# Autodesk Inventor assembly: ASY MSC 120  base frame
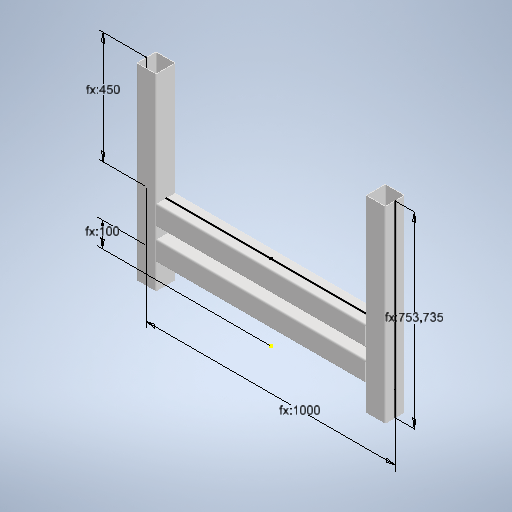
[picture p0: Inventor's stored thumbnail of the model, 512x512]
Saved by Autodesk Inventor 2025 (Build 290162010, 162A)
## iProperties
_SolveAssemblyDoc: Frame Generator Solve Assembly
_Version: 25.0.0
Created: 2024-06-27
Part Number: ASY MSC 120  base frame
Document SubType Name: Assembly
Designer: admin
Author: admin
## Documents named in this file (4)
- C:\Users\pokla\Documents\Inventor\Отстойник осветлитель\Manturovo_Se-clar-Gleb\Рама основания\ASY MSC 120  base frame.iam
- C:\Users\pokla\Documents\Inventor\Отстойник осветлитель\Manturovo_Se-clar-Gleb\Рама основания\MSC 100 base frame.ipt
- C:\Users\pokla\Documents\Inventor\Отстойник осветлитель\Manturovo_Se-clar-Gleb\Рама основания\ASY MSC 120  base frame\Frame\Frame 1719510697528.iam
- C:\Users\pokla\Documents\Inventor\Отстойник осветлитель\Manturovo_Se-clar-Gleb\Чертеж для парам. рамы.ipt
## Components (2 placed, 2 different names)
1. MSC 100 base frame:1
2. Frame 1719510697528:1 [sub-assembly]
## Named parameters: frame_1 = 403.7349 mm, frame_3 = 1689.31012 mm, frame_4 = 2332.09773 mm, frame_5 = 2974.88534 mm, Ширина_рамы = 1000 mm, Отступ_до_ниж_перекладины = 100 mm, Отступ_до_верх_перекладины = 450 mm, Шаг_опор_по_баку = 1000 mm, Движение_рамы_вперед_назад = 270 mm, frame_2 = 1046.52251 mm, frame_6 = 3617.67295 mm
